# Autodesk Inventor assembly: UpperArm
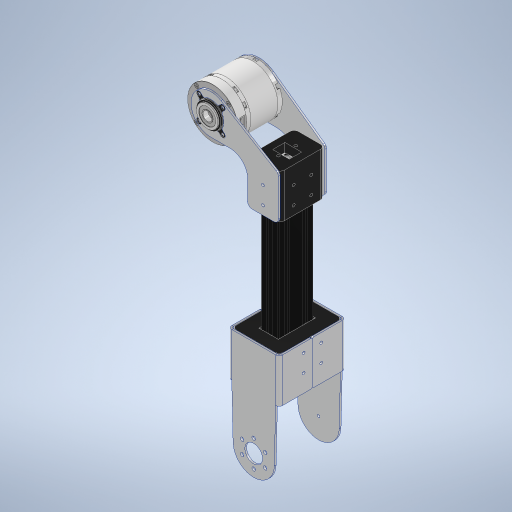
[picture p0: Inventor's stored thumbnail of the model, 512x512]
Saved by Autodesk Inventor 2024.3 (Build 283343010, 343A)
## iProperties
Created: 2025-05-20
Part Number: UpperArm
Document SubType Name: Assembly
Designer: kshau
Mass: 858.674 g
Surface Area: 2571.4 cm^2
Volume: 504.312 cm^3
Author: kshau
## Documents named in this file (13)
- C:\Users\kshau\Documents\inventor\Create_ViperX\Create_ViperX_ALOHA\UpperArm_Component\UpperArm.iam
- C:\Users\kshau\Documents\inventor\Create_ViperX\Create_ViperX_ALOHA\UpperArm_Component\upper_parameter.ipt
- C:\Users\kshau\Documents\inventor\Create_ViperX\Create_ViperX_ALOHA\UpperArm_Component\servoplate1_forR3.ipt
- C:\Users\kshau\Documents\inventor\Create_ViperX\Create_ViperX_ALOHA\UpperArm_Component\servoplate2_forR3.ipt
- C:\Users\kshau\Documents\inventor\Create_ViperX\Create_ViperX_ALOHA\UpperArm_Component\framefixpart1.ipt
- C:\Users\kshau\Documents\inventor\Create_ViperX\Create_ViperX_ALOHA\UpperArm_Component\framefixpart2.ipt
- C:\Users\kshau\Documents\inventor\Create_ViperX\Create_ViperX_ALOHA\NessesaryParts\HFSB5-2040-200\HFSB5-2040-200\HFSB5-2040-200.ipt
- C:\Users\kshau\Documents\inventor\Create_ViperX\Create_ViperX_ALOHA\Actuator\RS00\RS00\RS00.iam
- C:\Users\kshau\Documents\inventor\Create_ViperX\Create_ViperX_ALOHA\UpperArm_Component\servohorn_forR0.ipt
- C:\Users\kshau\Documents\inventor\Create_ViperX\Create_ViperX_ALOHA\UpperArm_Component\servohorn_support_forR0.ipt
- C:\Users\kshau\Documents\inventor\Create_ViperX\Create_ViperX_ALOHA\BasicParts\Bearing\NMB_RF2210X2HH\RF-2210X2HH.iam
- C:\Users\kshau\Documents\inventor\Create_ViperX\Create_ViperX_ALOHA\UpperArm_Component\upperarm_fixplate1_forR0.ipt
- C:\Users\kshau\Documents\inventor\Create_ViperX\Create_ViperX_ALOHA\UpperArm_Component\upperarm_fixplate2_forR0.ipt
## Components (12 placed, 12 different names)
1. upper_parameter:1
2. servoplate1_forR3:1 — フラッシュ:1, フラッシュ:2, メイト:1, 回転:1, フラッシュ:3
3. servoplate2_forR3:1 — フラッシュ:1, フラッシュ:2, メイト:1
4. framefixpart1:1 — 回転:1, フラッシュ:3, 回転:13, 回転:14
5. framefixpart2:1 — 回転:11, 回転:12, 回転:19, 回転:20, 回転:21, 回転:22
6. HFSB5-2040-200:1 — 回転:11, 回転:12, 回転:13, 回転:14
7. RS00:1 [sub-assembly] — 回転:17, 回転:18, メイト:2, 回転:23, 回転:24
8. servohorn_forR0:1 — 回転:17, 回転:18
9. servohorn_support_forR0:1 — メイト:3
10. RF-2210X2HH:1 [sub-assembly] — メイト:2, メイト:3
11. upperarm_fixplate1_forR0:1 — 回転:19, 回転:20, 回転:23, 回転:24
12. upperarm_fixplate2_forR0:1 — 回転:21, 回転:22
## Relationships (19: RevoluteJoint 13, Flush 3, Mate 3)
- フラッシュ:1 [Flush]: servoplate1_forR3:1 ↔ servoplate2_forR3:1
- フラッシュ:2 [Flush]: servoplate1_forR3:1 ↔ servoplate2_forR3:1
- メイト:1 [Mate]: servoplate1_forR3:1 ↔ servoplate2_forR3:1
- 回転:1 [RevoluteJoint]: servoplate1_forR3:1 ↔ framefixpart1:1
- フラッシュ:3 [Flush]: servoplate1_forR3:1 ↔ framefixpart1:1
- 回転:11 [RevoluteJoint]: framefixpart2:1 ↔ HFSB5-2040-200:1
- 回転:12 [RevoluteJoint]: framefixpart2:1 ↔ HFSB5-2040-200:1
- 回転:13 [RevoluteJoint]: framefixpart1:1 ↔ HFSB5-2040-200:1
- 回転:14 [RevoluteJoint]: framefixpart1:1 ↔ HFSB5-2040-200:1
- 回転:17 [RevoluteJoint]: RS00:1 ↔ servohorn_forR0:1
- 回転:18 [RevoluteJoint]: RS00:1 ↔ servohorn_forR0:1
- メイト:2 [Mate]: RS00:1 ↔ RF-2210X2HH:1
- メイト:3 [Mate]: servohorn_support_forR0:1 ↔ RF-2210X2HH:1
- 回転:19 [RevoluteJoint]: framefixpart2:1 ↔ upperarm_fixplate1_forR0:1
- 回転:20 [RevoluteJoint]: framefixpart2:1 ↔ upperarm_fixplate1_forR0:1
- 回転:21 [RevoluteJoint]: framefixpart2:1 ↔ upperarm_fixplate2_forR0:1
- 回転:22 [RevoluteJoint]: framefixpart2:1 ↔ upperarm_fixplate2_forR0:1
- 回転:23 [RevoluteJoint]: RS00:1 ↔ upperarm_fixplate1_forR0:1
- 回転:24 [RevoluteJoint]: RS00:1 ↔ upperarm_fixplate1_forR0:1
